# Autodesk Inventor assembly: Layer2Assembly
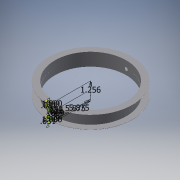
[picture p0: Inventor's stored thumbnail of the model, 180x180]
Saved by Autodesk Inventor 2017 (Build 210142000, 142)
## iProperties
Created: 2016-12-23
Part Number: Layer2Assembly
Document SubType Name: Assembly
Designer: David Kopala
Author: David Kopala
## Documents named in this file (3)
- \\Mac\Home\Documents\Drone\Drone\3D Models\Project\Chasis_02\Layer2Assembly.iam
- \\Mac\Home\Documents\Drone\Drone\3D Models\Project\Chasis_02\Layer2_Bottom.ipt
- \\Mac\Home\Documents\Drone\Drone\3D Models\Project\Chasis_02\Layer2_Top.ipt
## Components (2 placed, 2 different names)
1. Layer2_Bottom:1 — Insert:1, Flush:1
2. Layer2_Top:1 — Insert:1, Flush:1
## Relationships (2: Insert 1, Flush 1)
- Insert:1: Layer2_Bottom:1 ↔ Layer2_Top:1
- Flush:1: Layer2_Bottom:1 ↔ Layer2_Top:1
